# Autodesk Inventor assembly: 4K shield2
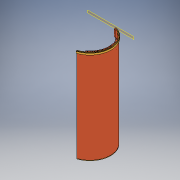
[picture p0: Inventor's stored thumbnail of the model, 180x180]
Saved by Autodesk Inventor 2018 (Build 220112000, 112)
## iProperties
Created: 2019-03-11
Part Number: 4K shield2
Document SubType Name: Assembly
Designer: Admin
Author: Admin
## Documents named in this file (6)
- C:\Users\Admin\Documents\Cryostat\CAD\4K shield2.iam
- C:\Users\Admin\Documents\Cryostat\CAD\4K sheild body2.ipt
- C:\Users\Admin\Documents\Cryostat\CAD\4K sheild rim3.ipt
- C:\Users\Admin\Documents\Cryostat\CAD\4K shield bottom.ipt
- C:\Users\Admin\Documents\Cryostat\CAD\4K shield cover.ipt
- C:\Users\Admin\Documents\Cryostat\CAD\4K adapter.ipt
## Components (12 placed, 5 different names)
1. 4K sheild body2:1 — Mate:1, Mate:2, Mate:3, Mate:4, Mate:9, Mate:10, Mate:11, Mate:12, Mate:13, Mate:14, Mate:15, Mate:16
2. 4K sheild rim3:1 — Mate:1, Mate:2, Flush:8
3. 4K shield bottom:1 — Mate:3, Mate:4, Mate:6, Mate:7, Mate:8
4. 4K shield cover:1 — Mate:6, Mate:7, Mate:8
5. 4K adapter:1 — Mate:10, Flush:3, Flush:7
6. 4K adapter:2 — Mate:12, Flush:4
7. 4K adapter:3 — Mate:15, Flush:7
8. 4K adapter:4 — Mate:16, Flush:1, Flush:4, Flush:8
9. 4K adapter:5 — Mate:9, Flush:5
10. 4K adapter:6 — Mate:11, Flush:6
11. 4K adapter:7 — Mate:13, Flush:2, Flush:3, Flush:6
12. 4K adapter:8 — Mate:14, Flush:1, Flush:2, Flush:5
## Relationships (23: Mate 15, Flush 8)
- Mate:1: 4K sheild body2:1 ↔ 4K sheild rim3:1
- Mate:2: 4K sheild body2:1 ↔ 4K sheild rim3:1
- Mate:3: 4K sheild body2:1 ↔ 4K shield bottom:1
- Mate:4: 4K sheild body2:1 ↔ 4K shield bottom:1
- Mate:6: 4K shield bottom:1 ↔ 4K shield cover:1
- Mate:7: 4K shield bottom:1 ↔ 4K shield cover:1
- Mate:8: 4K shield bottom:1 ↔ 4K shield cover:1
- Mate:9: 4K sheild body2:1 ↔ 4K adapter:5
- Mate:10: 4K sheild body2:1 ↔ 4K adapter:1
- Mate:11: 4K sheild body2:1 ↔ 4K adapter:6
- Mate:12: 4K sheild body2:1 ↔ 4K adapter:2
- Mate:13: 4K sheild body2:1 ↔ 4K adapter:7
- Mate:14: 4K sheild body2:1 ↔ 4K adapter:8
- Mate:15: 4K sheild body2:1 ↔ 4K adapter:3
- Mate:16: 4K sheild body2:1 ↔ 4K adapter:4
- Flush:1: 4K adapter:4 ↔ 4K adapter:8
- Flush:2: 4K adapter:7 ↔ 4K adapter:8
- Flush:3: 4K adapter:1 ↔ 4K adapter:7
- Flush:4: 4K adapter:2 ↔ 4K adapter:4
- Flush:5: 4K adapter:5 ↔ 4K adapter:8
- Flush:6: 4K adapter:6 ↔ 4K adapter:7
- Flush:7: 4K adapter:1 ↔ 4K adapter:3
- Flush:8: 4K sheild rim3:1 ↔ 4K adapter:4
